# Autodesk Inventor assembly: detector_chamber4
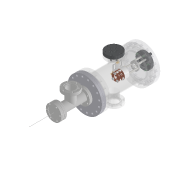
[picture p0: Inventor's stored thumbnail of the model, 180x180]
Saved by Autodesk Inventor 2020 (Build 240168000, 168)
## iProperties
Created: 2022-09-29
Part Number: detector_chamber4
Document SubType Name: Assembly
Designer: robco
Author: robco
## Documents named in this file (11)
- C:\Physics\nEXO\CAD_modelling\Ba-tagging\PIPS\alternative1\detector_chamber4.iam
- C:\Physics\nEXO\CAD_modelling\standard_parts\feedthroughs\iftbg022033_PIPStapped.ipt
- C:\Physics\nEXO\CAD_modelling\Ba-tagging\PIPS\alternative1\detector_alt3.iam
- C:\Physics\nEXO\CAD_modelling\Ba-tagging\PIPS\alternative1\wavelength_shifter.ipt
- C:\Physics\nEXO\CAD_modelling\Ba-tagging\PIPS\alternative1\MicroFJ-SMA-60035_board.iam
- C:\Physics\nEXO\CAD_modelling\standard_parts\crosses\c-0600-275.iam
- C:\Physics\nEXO\CAD_modelling\standard_parts\reducers\rf600x275.ipt
- C:\Physics\nEXO\CAD_modelling\standard_parts\tee\t-0275.iam
- C:\Physics\nEXO\raad_stuff\mount\boil-2.iam
- C:\Physics\nEXO\CAD_modelling\standard_parts\feedthroughs\ifdcg042013.ipt
- C:\Physics\nEXO\CAD_modelling\Ba-tagging\PIPS\alternative1\teflon_rings.ipt
## Components (12 placed, 10 different names)
1. c-0600-275:1 [sub-assembly] — Mate:23, Mate:24, Mate:27, Mate:28, Mate:29, Mate:33, Mate:34, Angle:3, Mate:35, Mate:36
2. rf600x275:1 — Mate:23, Mate:24, Mate:25, Mate:26
3. iftbg022033_PIPStapped:1 — Mate:17, Mate:18, Mate:20, Mate:25, Mate:26
4. detector_alt3:1 [sub-assembly] — Mate:17, Mate:18, Mate:20, Mate:37, Mate:38
5. wavelength_shifter:1
6. MicroFJ-SMA-60035_board:1 [sub-assembly] — Angle:1, Angle:2
7. rf600x275:2 — Mate:27, Mate:28, Mate:30
8. t-0275:1 [sub-assembly] — Mate:29, Mate:30, Mate:31, Mate:32
9. boil-2:1 [sub-assembly] — Mate:31, Mate:32
10. t-0275:2 [sub-assembly] — Mate:33, Mate:34, Angle:3
11. ifdcg042013:1 — Mate:35, Mate:36
12. teflon_rings:1 — Mate:37, Mate:38
## Relationships (23: Mate 20, Angle 3)
- Mate:17: iftbg022033_PIPStapped:1 ↔ detector_alt3:1
- Mate:18: iftbg022033_PIPStapped:1 ↔ detector_alt3:1
- Mate:20: iftbg022033_PIPStapped:1 ↔ detector_alt3:1
- [Mate]: c-0600-275:1 ↔ wavelength_shifter:1
- Angle:1 (0 deg): MicroFJ-SMA-60035_board:1
- Angle:2 (0 deg): MicroFJ-SMA-60035_board:1
- Mate:23: c-0600-275:1 ↔ rf600x275:1
- Mate:24: c-0600-275:1 ↔ rf600x275:1
- Mate:25: rf600x275:1 ↔ iftbg022033_PIPStapped:1
- Mate:26: rf600x275:1 ↔ iftbg022033_PIPStapped:1
- Mate:27: c-0600-275:1 ↔ rf600x275:2
- Mate:28: c-0600-275:1 ↔ rf600x275:2
- Mate:29: c-0600-275:1 ↔ t-0275:1
- Mate:30: rf600x275:2 ↔ t-0275:1
- Mate:31: t-0275:1 ↔ boil-2:1
- Mate:32: t-0275:1 ↔ boil-2:1
- Mate:33: c-0600-275:1 ↔ t-0275:2
- Mate:34: c-0600-275:1 ↔ t-0275:2
- Angle:3 (0 deg): c-0600-275:1 ↔ t-0275:2
- Mate:35: c-0600-275:1 ↔ ifdcg042013:1
- Mate:36: c-0600-275:1 ↔ ifdcg042013:1
- Mate:37: detector_alt3:1 ↔ teflon_rings:1
- Mate:38 (2 mm): detector_alt3:1 ↔ teflon_rings:1
